# Autodesk Inventor assembly: Assembly1
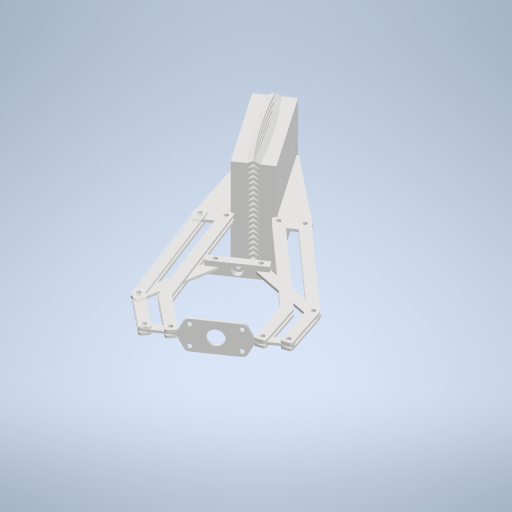
[picture p0: Inventor's stored thumbnail of the model, 512x512]
Saved by Autodesk Inventor 2023 (Build 270158000, 158)
## iProperties
Created: 2023-03-02
Part Number: Assembly1
Document SubType Name: Assembly
Designer: Gabriel - T3 CAD
Author: Gabriel - T3 CAD
## Documents named in this file (15)
- C:\Users\Gabriel - T3 CAD\Documents\GitHub\T3-CAD\New folder\New folder\Assembly1.iam
- C:\Users\Gabriel - T3 CAD\Documents\GitHub\T3-CAD\New folder\New folder\Outer Gripper Bar.ipt
- C:\Users\Gabriel - T3 CAD\Documents\GitHub\T3-CAD\New folder\New folder\Inner Gripper Bar.ipt
- C:\Users\Gabriel - T3 CAD\Documents\GitHub\T3-CAD\New folder\Connector.ipt
- C:\Users\Gabriel - T3 CAD\Documents\GitHub\T3-CAD\New folder\Face Plate.ipt
- C:\Users\Gabriel - T3 CAD\Documents\GitHub\T3-CAD\New folder\Gripper plate.ipt
- C:\Users\Gabriel - T3 CAD\Documents\GitHub\T3-CAD\New folder\Gripper triangle.ipt
- C:\Users\Gabriel - T3 CAD\Documents\GitHub\T3-CAD\Current Season CAD\Swerve-DriveTrain-V2.1 (LongBot)\Potential new gripper\Gripper plate v2.ipt
- C:\Users\Gabriel - T3 CAD\Documents\GitHub\T3-CAD\New folder\Pusher.ipt
- C:\Users\Gabriel - T3 CAD\Documents\GitHub\T3-CAD\New folder\New folder\Outer Gripper Bar_MIR.ipt
- C:\Users\Gabriel - T3 CAD\Documents\GitHub\T3-CAD\New folder\New folder\Inner Gripper Bar_MIR.ipt
- C:\Users\Gabriel - T3 CAD\Documents\GitHub\T3-CAD\New folder\Gripper plate_MIR1.ipt
- C:\Users\Gabriel - T3 CAD\Documents\GitHub\T3-CAD\New folder\Gripper triangle_MIR1.ipt
- C:\Users\Gabriel - T3 CAD\Documents\GitHub\T3-CAD\Current Season CAD\Swerve-DriveTrain-V2.1 (LongBot)\Potential new gripper\Gripper plate v2_MIR1.ipt
- C:\Users\Gabriel - T3 CAD\Documents\GitHub\T3-CAD\New folder\Pusher_MIR1.ipt
## Components (18 placed, 14 different names)
1. Outer Gripper Bar:4 — Rotational:2, Rotational:4
2. Outer Gripper Bar:5 — Rotational:1, Rotational:3, Rotational:8
3. Inner Gripper Bar:1 — Rotational:6, Rotational:9, Rotational:10
4. Connector:1 — Rotational:7, Rotational:16, Cylindrical:1
5. Face Plate:1 — Rotational:3, Rotational:4, Rotational:5, Rotational:6, Cylindrical:1, Rotational:18, Rotational:19, Rotational:20
6. Gripper plate:1 — Rigid:1, Rigid:4
7. Gripper triangle:1 — Rigid:1, Rotational:8, Rotational:10
8. Gripper plate v2:1 — Rigid:4
9. Pusher:2 — Rotational:1, Rotational:2, Rotational:7
10. Inner Gripper Bar:5 — Rotational:5, Rotational:9
11. Outer Gripper Bar_MIR:1 — Rotational:13, Rotational:17
12. Outer Gripper Bar_MIR:2 — Rotational:12, Rotational:14, Rotational:17, Rotational:18
13. Inner Gripper Bar_MIR:1 — Rotational:11, Rotational:15, Rotational:19
14. Gripper plate_MIR1:1 — Rigid:5, Rigid:6
15. Gripper triangle_MIR1:1 — Rotational:11, Rotational:12, Rigid:5
16. Gripper plate v2_MIR1:1 — Rigid:6
17. Pusher_MIR1:1 — Rotational:13, Rotational:14, Rotational:16
18. Inner Gripper Bar_MIR:2 — Rotational:15, Rotational:20
## Relationships (25: RevoluteJoint 20, WeldJoint 4, CylindricalJoint 1)
- Rigid:1 [WeldJoint]: Gripper plate:1 ↔ Gripper triangle:1
- Rigid:4 [WeldJoint]: Gripper plate:1 ↔ Gripper plate v2:1
- Rotational:1 [RevoluteJoint]: Outer Gripper Bar:5 ↔ Pusher:2
- Rotational:2 [RevoluteJoint]: Outer Gripper Bar:4 ↔ Pusher:2
- Rotational:3 [RevoluteJoint]: Outer Gripper Bar:5 ↔ Face Plate:1
- Rotational:4 [RevoluteJoint]: Outer Gripper Bar:4 ↔ Face Plate:1
- Rotational:5 [RevoluteJoint]: Face Plate:1 ↔ Inner Gripper Bar:5
- Rotational:6 [RevoluteJoint]: Inner Gripper Bar:1 ↔ Face Plate:1
- Rotational:7 [RevoluteJoint]: Connector:1 ↔ Pusher:2
- Rotational:8 [RevoluteJoint]: Outer Gripper Bar:5 ↔ Gripper triangle:1
- Rotational:9 [RevoluteJoint] (3.175 mm): Inner Gripper Bar:1 ↔ Inner Gripper Bar:5
- Rotational:10 [RevoluteJoint]: Inner Gripper Bar:1 ↔ Gripper triangle:1
- Rotational:11 [RevoluteJoint]: Inner Gripper Bar_MIR:1 ↔ Gripper triangle_MIR1:1
- Rotational:12 [RevoluteJoint]: Outer Gripper Bar_MIR:2 ↔ Gripper triangle_MIR1:1
- Rigid:5 [WeldJoint]: Gripper plate_MIR1:1 ↔ Gripper triangle_MIR1:1
- Rigid:6 [WeldJoint]: Gripper plate_MIR1:1 ↔ Gripper plate v2_MIR1:1
- Rotational:13 [RevoluteJoint]: Outer Gripper Bar_MIR:1 ↔ Pusher_MIR1:1
- Rotational:14 [RevoluteJoint]: Outer Gripper Bar_MIR:2 ↔ Pusher_MIR1:1
- Rotational:15 [RevoluteJoint] (-3.175 mm): Inner Gripper Bar_MIR:1 ↔ Inner Gripper Bar_MIR:2
- Rotational:16 [RevoluteJoint]: Connector:1 ↔ Pusher_MIR1:1
- Cylindrical:1: Connector:1 ↔ Face Plate:1
- Rotational:17 [RevoluteJoint] (3.175 mm): Outer Gripper Bar_MIR:1 ↔ Outer Gripper Bar_MIR:2
- Rotational:18 [RevoluteJoint]: Face Plate:1 ↔ Outer Gripper Bar_MIR:2
- Rotational:19 [RevoluteJoint]: Face Plate:1 ↔ Inner Gripper Bar_MIR:1
- Rotational:20 [RevoluteJoint] (3.175 mm): Face Plate:1 ↔ Inner Gripper Bar_MIR:2
